# Autodesk Inventor assembly: HbCircuit
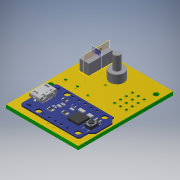
[picture p0: Inventor's stored thumbnail of the model, 180x180]
Saved by Autodesk Inventor 2017 (Build 210142000, 142)
## iProperties
Part Number: HbCircuit
Material: 一般
Document SubType Name: Assembly
Designer: sktom
Author: sktom
## Documents named in this file (5)
- D:\OneDrive\CAD\MAJ\hackberry\HACKberry-hardware\3D_69%inlength\Inventor\HbHandForChild\HbCircuit\HbCircuit.iam
- D:\OneDrive\CAD\MAJ\hackberry\HACKberry-hardware\3D_69%inlength\Inventor\HbHandForChild\HbCircuit\HbSizeS.ipt
- D:\OneDrive\CAD\MAJ\hackberry\HACKberry-hardware\3D_69%inlength\Inventor\HbHandForChild\HbCircuit\SS-12SDP2.ipt
- D:\OneDrive\CAD\MAJ\hackberry\HACKberry-hardware\3D_69%inlength\Inventor\HbHandForChild\HbCircuit\trinket 5V.ipt
- D:\OneDrive\CAD\MAJ\hackberry\HACKberry-hardware\3D_69%inlength\Inventor\HbHandForChild\HbCircuit\SKRGAQD010.ipt
## Components (4 placed, 4 different names)
1. HbSizeS:1 — 挿入:1, 挿入:2, 挿入:3
2. SS-12SDP2:1 — 挿入:1
3. trinket 5V:1 — 挿入:3
4. SKRGAQD010:1 — 挿入:2
## Relationships (3: Insert 3)
- 挿入:1 [Insert]: HbSizeS:1 ↔ SS-12SDP2:1
- 挿入:2 [Insert]: HbSizeS:1 ↔ SKRGAQD010:1
- 挿入:3 [Insert] (1 mm): HbSizeS:1 ↔ trinket 5V:1
